# Autodesk Inventor assembly: Assembly
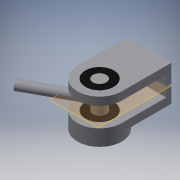
[picture p0: Inventor's stored thumbnail of the model, 180x180]
Saved by Autodesk Inventor 2017 (Build 210142000, 142)
## iProperties
Created: 2017-08-06
Part Number: Assembly
Document SubType Name: Assembly
Designer: Bardo91
Author: Bardo91
## Documents named in this file (5)
- D:\programming\cad_hexacopter\positioner\Assembly.iam
- D:\programming\cad_hexacopter\positioner\baseRotor1.ipt
- D:\programming\cad_hexacopter\positioner\rodamiento15_32.ipt
- D:\programming\cad_hexacopter\positioner\rotor1.ipt
- D:\programming\cad_hexacopter\positioner\potentiometer.ipt
## Components (5 placed, 4 different names)
1. baseRotor1:1 — Mate:1, Mate:2, Mate:3, Flush:1, Mate:9
2. rodamiento15_32:1 — Mate:1, Mate:2
3. rodamiento15_32:2 — Mate:3, Flush:1, Mate:8
4. rotor1:1 — Mate:4, Mate:5, Mate:6, Mate:8
5. potentiometer:1 — Mate:4, Mate:5, Mate:6, Mate:9
## Relationships (9: Mate 8, Flush 1)
- Mate:1: baseRotor1:1 ↔ rodamiento15_32:1
- Mate:2: baseRotor1:1 ↔ rodamiento15_32:1
- Mate:3: baseRotor1:1 ↔ rodamiento15_32:2
- Flush:1: baseRotor1:1 ↔ rodamiento15_32:2
- Mate:4: rotor1:1 ↔ potentiometer:1
- Mate:5: rotor1:1 ↔ potentiometer:1
- Mate:6: rotor1:1 ↔ potentiometer:1
- Mate:8: rodamiento15_32:2 ↔ rotor1:1
- Mate:9: baseRotor1:1 ↔ potentiometer:1
